# Autodesk Inventor assembly: Test mechanum wheel drive train
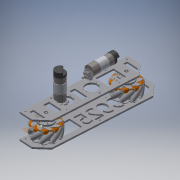
[picture p0: Inventor's stored thumbnail of the model, 180x180]
Saved by Autodesk Inventor 2017 (Build 210142000, 142)
## iProperties
Created: 2017-08-02
Part Number: Test mechanum wheel drive train
Document SubType Name: Assembly
Designer: User
Author: User
## Documents named in this file (5)
- C:\Robotics\CAD\2016-17_CAD\Test mechanum wheel drive train.iam
- C:\Robotics\CAD\2016-17_CAD\DriveTrain\DrainTrainPlate2.0LeftOutside.iam
- C:\Robotics\CAD\2016-17_CAD\DriveTrain\wheel sub assembly mechanum wheels .iam
- C:\Robotics\CAD\2016-17_CAD\DriveTrain\DriveTrainPlate2.0LeftInside.ipt
- C:\Robotics\CAD\2016-17_CAD\DriveTrain\motor sub assembley.iam
## Components (6 placed, 4 different names)
1. DrainTrainPlate2.0LeftOutside:1 [sub-assembly] — Mate:3, Mate:4, Mate:5, Mate:8
2. wheel sub assembly mechanum wheels :1 [sub-assembly] — Mate:6, Mate:7, Mate:8, Flush:1
3. wheel sub assembly mechanum wheels :2 [sub-assembly] — Mate:1, Mate:2, Mate:3, Mate:4, Mate:5
4. DriveTrainPlate2.0LeftInside:1 — Mate:1, Mate:2, Mate:6, Mate:7
5. motor sub assembley:1 [sub-assembly] — Flush:1
6. motor sub assembley:2 [sub-assembly]
## Relationships (9: Mate 8, Flush 1)
- Mate:1 (6.35 mm): wheel sub assembly mechanum wheels :2 ↔ DriveTrainPlate2.0LeftInside:1
- Mate:2: wheel sub assembly mechanum wheels :2 ↔ DriveTrainPlate2.0LeftInside:1
- Mate:3: DrainTrainPlate2.0LeftOutside:1 ↔ wheel sub assembly mechanum wheels :2
- Mate:4: DrainTrainPlate2.0LeftOutside:1 ↔ wheel sub assembly mechanum wheels :2
- Mate:5: DrainTrainPlate2.0LeftOutside:1 ↔ wheel sub assembly mechanum wheels :2
- Mate:6 (6.35 mm): wheel sub assembly mechanum wheels :1 ↔ DriveTrainPlate2.0LeftInside:1
- Mate:7: wheel sub assembly mechanum wheels :1 ↔ DriveTrainPlate2.0LeftInside:1
- Mate:8: DrainTrainPlate2.0LeftOutside:1 ↔ wheel sub assembly mechanum wheels :1
- Flush:1: wheel sub assembly mechanum wheels :1 ↔ motor sub assembley:1
